# Autodesk Inventor assembly: Tasma2
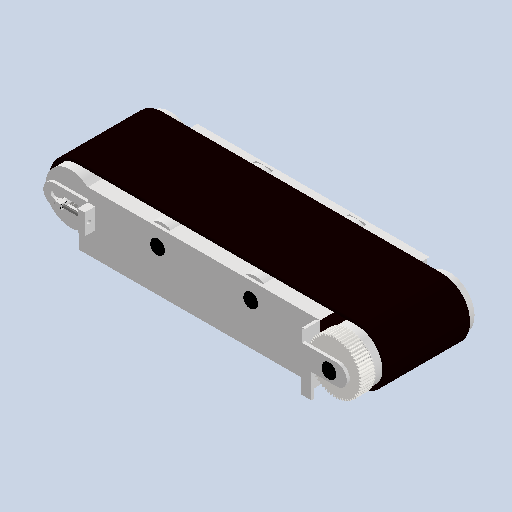
[picture p0: Inventor's stored thumbnail of the model, 512x512]
Saved by Autodesk Inventor 2022 (Build 260153000, 153)
## iProperties
Created: 2023-04-25
Part Number: Tasma2
Document SubType Name: Assembly
Designer: nosal
Author: nosal
## Documents named in this file (11)
- C:\Users\nosal\OneDrive\Pulpit\projekty 3d\Inżynierka\Tasma2\Tasma2.iam
- C:\Users\nosal\OneDrive\Pulpit\projekty 3d\Inżynierka\Tasma2\wał_tylni2.ipt
- C:\Users\nosal\OneDrive\Pulpit\projekty 3d\Inżynierka\Tasma2\wały_sr.ipt
- C:\Users\nosal\OneDrive\Pulpit\projekty 3d\Inżynierka\Tasma2\wal_sr_tyl.ipt
- C:\Users\nosal\OneDrive\Pulpit\projekty 3d\Inżynierka\Tasma2\Design Accelerator\Łożysko1.iam
- C:\Users\nosal\OneDrive\Pulpit\projekty 3d\Inżynierka\Tasma2\pastran.ipt
- C:\Users\nosal\OneDrive\Pulpit\projekty 3d\Inżynierka\Tasma2\Podstawa.ipt
- C:\Users\nosal\OneDrive\Pulpit\projekty 3d\Inżynierka\Tasma2\Przekładnia walcowa26.ipt
- C:\Users\nosal\OneDrive\Pulpit\projekty 3d\Inżynierka\Tasma2\patyk.ipt
- C:\Users\nosal\OneDrive\Pulpit\projekty 3d\Inżynierka\Tasma2\patyk2.ipt
- C:\Users\nosal\OneDrive\Dokumenty\Inventor\Content Center Files\R2022\pl-PL\IS 1366\IS 1366 - M4 x 40.ipt
## Components (21 placed, 10 different names)
1. wał_tylni2:1 — Zestawiające:1, Zestawiające:6, Sztywne:1
2. wał_tylni2:2 — Zestawiające:4, Zestawiające:5, Sztywne:4
3. wały_sr:1 — Zestawiające:2, Zestawiające:7, Obrotowe:3
4. wały_sr:2 — Zestawiające:3, Zestawiające:8, Obrotowe:4
5. wal_sr_tyl:1 — Sztywne:1, Sztywne:5, Sztywne:6
6. Łożysko:1 [sub-assembly] — Zestawiające:2
7. Łożysko:2 [sub-assembly] — Zestawiające:3
8. Łożysko:3 [sub-assembly] — Zestawiające:4, Sztywne:3
9. Łożysko:4 [sub-assembly] — Zestawiające:5
10. Łożysko:5 [sub-assembly] — Zestawiające:6
11. Łożysko:6 [sub-assembly] — Zestawiające:7
12. Łożysko:7 [sub-assembly] — Zestawiające:8
13. Łożysko:8 [sub-assembly] — Zestawiające:1
14. pastran:1
15. Podstawa:1 — Sztywne:2, Obrotowe:1, Obrotowe:2
16. Przekładnia walcowa2:1 — Sztywne:3
17. patyk:1 — Sztywne:2, Obrotowe:3
18. patyk:2 — Obrotowe:1, Obrotowe:4
19. patyk2:1 — Obrotowe:2, Sztywne:4
20. IS 1366 M4 x 40:1 — Sztywne:5
21. IS 1366 M4 x 40:2 — Sztywne:6
## Relationships (18: Mate 8, WeldJoint 6, RevoluteJoint 4)
- Zestawiające:1 [Mate]: wał_tylni2:1 ↔ Łożysko:8
- Zestawiające:2 [Mate]: wały_sr:1 ↔ Łożysko:1
- Zestawiające:3 [Mate]: wały_sr:2 ↔ Łożysko:2
- Zestawiające:4 [Mate]: wał_tylni2:2 ↔ Łożysko:3
- Zestawiające:5 [Mate]: wał_tylni2:2 ↔ Łożysko:4
- Zestawiające:6 [Mate]: wał_tylni2:1 ↔ Łożysko:5
- Zestawiające:7 [Mate]: wały_sr:1 ↔ Łożysko:6
- Zestawiające:8 [Mate]: wały_sr:2 ↔ Łożysko:7
- Sztywne:1 [WeldJoint] (-150.5 mm): wał_tylni2:1 ↔ wal_sr_tyl:1
- Sztywne:2 [WeldJoint] (-0.5 mm): Podstawa:1 ↔ patyk:1
- Obrotowe:1 [RevoluteJoint] (-0.5 mm): Podstawa:1 ↔ patyk:2
- Obrotowe:2 [RevoluteJoint] (-0.5 mm): Podstawa:1 ↔ patyk2:1
- Obrotowe:3 [RevoluteJoint]: wały_sr:1 ↔ patyk:1
- Obrotowe:4 [RevoluteJoint]: wały_sr:2 ↔ patyk:2
- Sztywne:3 [WeldJoint]: Łożysko:3 ↔ Przekładnia walcowa2:1
- Sztywne:4 [WeldJoint] (10.5 mm): wał_tylni2:2 ↔ patyk2:1
- Sztywne:5 [WeldJoint] (-13 mm): wal_sr_tyl:1 ↔ IS 1366 M4 x 40:1
- Sztywne:6 [WeldJoint] (-21 mm): wal_sr_tyl:1 ↔ IS 1366 M4 x 40:2
